# Autodesk Inventor assembly: Left-X-linear bearing shroud
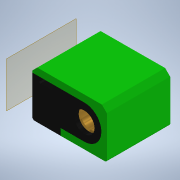
[picture p0: Inventor's stored thumbnail of the model, 180x180]
Saved by Autodesk Inventor 2020 (Build 240168000, 168)
## iProperties
Created: 2021-02-25
Part Number: Left-X-linear bearing shroud
Document SubType Name: Assembly
Designer: AOB
Mass: 35.4085 g
Surface Area: 103.275 cm^2
Volume: 12.7597 cm^3
Density: 2.77502 g/cm^3
Author: AOB
## Documents named in this file (4)
- C:\Users\marti\Documents\Inventor\ProjectBoron\ultimate boron\Left-X-linear bearing shroud.iam
- C:\Users\marti\Documents\Inventor\ProjectBoron\ultimate boron\Left-X-linear bearing shroud-B.ipt
- C:\Users\marti\Documents\Inventor\ProjectBoron\ultimate boron\Left-X-linear bearing shroud-A.ipt
- C:\Users\marti\Documents\Inventor\ProjectBoron\ultimate boron\Left-lm8uu-graphite1.ipt
## Components (3 placed, 3 different names)
1. Left-X-linear bearing shroud-B:1 — Flush:1, Rigid:1
2. Left-X-linear bearing shroud-A:1 — Mate:2, Mate:1, Flush:1, Flush:2, Rigid:1
3. Left-lm8uu-graphite1:1 — Mate:2, Mate:1
## Relationships (5: Mate 2, Flush 2, WeldJoint 1)
- Mate:2: Left-X-linear bearing shroud-A:1 ↔ Left-lm8uu-graphite1:1
- Mate:1: Left-X-linear bearing shroud-A:1 ↔ Left-lm8uu-graphite1:1
- Flush:1: Left-X-linear bearing shroud-B:1 ↔ Left-X-linear bearing shroud-A:1
- Flush:2 (10 mm): Left-X-linear bearing shroud-A:1
- Rigid:1 [WeldJoint]: Left-X-linear bearing shroud-B:1 ↔ Left-X-linear bearing shroud-A:1
